# Autodesk Inventor assembly: StorageAssembly.ver3-1111-2020
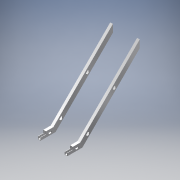
[picture p0: Inventor's stored thumbnail of the model, 180x180]
Saved by Autodesk Inventor 2018 (Build 220112000, 112)
## iProperties
Created: 2020-01-21
Part Number: StorageAssembly.ver3-1111-2020
Document SubType Name: Assembly
Designer: Power Hawks CADD
Author: Power Hawks CADD
## Documents named in this file (3)
- E:\GrabCAD\Power Hawks CAD\2020 Infinite Recharge\Storage\Assemblies\StorageAssembly.ver3-1111-2020.iam
- E:\GrabCAD\Power Hawks CAD\2020 Infinite Recharge\Shooting\Parts\AngleBrace.ver1-1111-2020.ipt
- E:\GrabCAD\Power Hawks CAD\2020 Infinite Recharge\Storage\Parts\BottomStorageSupport.ver1-1111-2020.ipt
## Components (4 placed, 2 different names)
1. AngleBrace.ver1-1111-2020:1 — Flush:3, Flush:5, Mate:4, Mate:5
2. BottomStorageSupport.ver1-1111-2020:1 — Flush:3, Flush:6, Mate:5
3. BottomStorageSupport.ver1-1111-2020:2 — Flush:4, Flush:6, Mate:6
4. AngleBrace.ver1-1111-2020:2 — Flush:4, Flush:5, Mate:4, Mate:6
## Relationships (9: Flush 6, Mate 3)
- [Flush]: AngleBrace.ver1-1111-2020:1 ↔ BottomStorageSupport.ver1-1111-2020:1
- [Flush]: BottomStorageSupport.ver1-1111-2020:2 ↔ AngleBrace.ver1-1111-2020:2
- Flush:3: AngleBrace.ver1-1111-2020:1 ↔ BottomStorageSupport.ver1-1111-2020:1
- Flush:4: BottomStorageSupport.ver1-1111-2020:2 ↔ AngleBrace.ver1-1111-2020:2
- Flush:5: AngleBrace.ver1-1111-2020:1 ↔ AngleBrace.ver1-1111-2020:2
- Flush:6: BottomStorageSupport.ver1-1111-2020:1 ↔ BottomStorageSupport.ver1-1111-2020:2
- Mate:4 (228.6 mm): AngleBrace.ver1-1111-2020:1 ↔ AngleBrace.ver1-1111-2020:2
- Mate:5: AngleBrace.ver1-1111-2020:1 ↔ BottomStorageSupport.ver1-1111-2020:1
- Mate:6: BottomStorageSupport.ver1-1111-2020:2 ↔ AngleBrace.ver1-1111-2020:2
